# Autodesk Inventor assembly: MR126ZZ
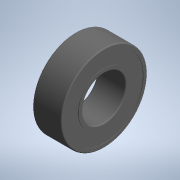
[picture p0: Inventor's stored thumbnail of the model, 180x180]
Saved by Autodesk Inventor 2022.3 (Build 263350000, 350)
## iProperties
Part Number: MR126ZZ
Catalog Web Link: www.cadenas.de
Description: Shielded Type ZZ-ZZS-
Vendor: NSK_RB
Document SubType Name: Assembly
Designer: partserver
Manufacturer: NSK_RB
Mass: 1.74 g
Surface Area: 9.09475 cm^2
Volume: 0.233443 cm^3
Density: 7.45365 g/cm^3
Category: PARTsolutions
Company: NSK_RB
PSOL_IDENT_0: {$CADENAS_DATA\23d-libs\nsk_rb\roller_bearings\deep_groove_bb\exstra_small_miniatur_bb\metric_design
PSOL_IDENT_1: \shielded_type_zz_zzs_asmtab.prj},174 {VTYP=3D},{STYP=ASSTAB},{NB=MR126ZZ},{LINA=MR126ZZ},{NN=Shield
PSOL_IDENT_2: ed Type ZZ-ZZS},{DATE=16.07.2021 00:25:30},{GEOMDATE=14.01.2008},{VERSION=},{LINEID=590},{WBVAR=},{W
PSOL_IDENT_3: BNUMERIC=}  {NB=MR126ZZ},{LINA=MR126ZZ},{KT=DUMMY},{IDNR=},{STAN=Standard},{ORDER=MR126ZZ},{SD=6.0},
PSOL_IDENT_4: {X=6.0},{DI1=7.73},{DI2=7.20},{SDE1=10.19},{SDE2=10.90},{D=12},{DD=12},{B=0.0},{B1=4.0},{R=0.00},{R1=
PSOL_IDENT_5: 0.15},{CR1=715},{COR1=292},{CR2=73},{COR2=30.0},{LG=43000},{LO=50000},{DA=0.0},{DB=7.2},{DA1=0.0},{D
PSOL_IDENT_6: B1=10.9},{RA=0.00},{RB=0.15},{MASS=1.74},{SC=1},{PPATH=shielded_type_zz_zzs_asmtpl.prj}
NB: MR126ZZ
NN: Shielded Type ZZ-ZZS
NBSYN: $ORDER.
LINA: MR126ZZ
CATALOG: NSK Rolling Bearing
STAN: Standard
ORDER: MR126ZZ
SD: 6
D: 12
B1: 4
R1: 0.15
CR1: 715
COR1: 292
CR2: 73
COR2: 30
LG: 43000
DB: 7.2
DB1: 10.9
RB: 0.15
MASS: 1.74
SUPPLIER: NSK_RB
ARTICLENO: MR126ZZ
BOMINFO: MR126ZZ
CREATOR: CADENAS GmbH
Title: MR126ZZ
Author: Cadenas PARTsolutions
## Documents named in this file (6)
- C:\Users\YusukeKunita\Documents\GrabCAD\Development\BasicParts\Bearing\NSK_RB_MR126ZZ\MR126ZZ.iam
- C:\Users\YusukeKunita\Documents\GrabCAD\Development\BasicParts\Bearing\NSK_RB_MR126ZZ\MR126ZZ Outer Ring.ipt
- C:\Users\YusukeKunita\Documents\GrabCAD\Development\BasicParts\Bearing\NSK_RB_MR126ZZ\MR126ZZ Inner Ring.ipt
- C:\Users\YusukeKunita\Documents\GrabCAD\Development\BasicParts\Bearing\NSK_RB_MR126ZZ\MR126ZZ Shield1.ipt
- C:\Users\YusukeKunita\Documents\GrabCAD\Development\BasicParts\Bearing\NSK_RB_MR126ZZ\MR126ZZ Ball.ipt
- C:\Users\YusukeKunita\Documents\GrabCAD\Development\BasicParts\Bearing\NSK_RB_MR126ZZ\MR126ZZ Shield2.ipt
## Components (16 placed, 5 different names)
1. MR126ZZ Outer Ring:1 — ip_st_or_1_XY@1 <-> ip_st_ir_1a_XY@2, ip_st_or_1_Z@1 <-> ip_st_ir_1a_Z@2, ip_st_or_1_YZ@1 <-> ip_st_ir_1a_YZ@2, ip_st_or_2_XY@1 <-> ip_st_s2_XY@16, ip_st_or_2_Z@1 <-> ip_st_s2_Z@16, ip_st_or_2_YZ@1 <-> ip_st_s2_YZ@16
2. MR126ZZ Inner Ring:1 — ip_st_or_1_XY@1 <-> ip_st_ir_1a_XY@2, ip_st_or_1_Z@1 <-> ip_st_ir_1a_Z@2, ip_st_or_1_YZ@1 <-> ip_st_ir_1a_YZ@2, ip_st_ir_2a_XY@2 <-> ip_st_s1_XY@3, ip_st_ir_2a_Z@2 <-> ip_st_s1_Z@3, ip_st_ir_2a_YZ@2 <-> ip_st_s1_YZ@3, ip_st_ir_1_1_XY@2 <-> ip_st_b_XY@4, ip_st_ir_1_1_Z@2 <-> ip_st_b_Z@4, ip_st_ir_1_1_YZ@2 <-> ip_st_b_YZ@4, ip_st_ir_1_2_XY@2 <-> ip_st_b_XY@5, ip_st_ir_1_2_Z@2 <-> ip_st_b_Z@5, ip_st_ir_1_2_YZ@2 <-> ip_st_b_YZ@5, ip_st_ir_1_3_XY@2 <-> ip_st_b_XY@6, ip_st_ir_1_3_Z@2 <-> ip_st_b_Z@6, ip_st_ir_1_3_YZ@2 <-> ip_st_b_YZ@6, ip_st_ir_1_4_XY@2 <-> ip_st_b_XY@7, ip_st_ir_1_4_Z@2 <-> ip_st_b_Z@7, ip_st_ir_1_4_YZ@2 <-> ip_st_b_YZ@7, ip_st_ir_1_5_XY@2 <-> ip_st_b_XY@8, ip_st_ir_1_5_Z@2 <-> ip_st_b_Z@8, ip_st_ir_1_5_YZ@2 <-> ip_st_b_YZ@8, ip_st_ir_1_6_XY@2 <-> ip_st_b_XY@9, ip_st_ir_1_6_Z@2 <-> ip_st_b_Z@9, ip_st_ir_1_6_YZ@2 <-> ip_st_b_YZ@9, ip_st_ir_1_7_XY@2 <-> ip_st_b_XY@10, ip_st_ir_1_7_Z@2 <-> ip_st_b_Z@10, ip_st_ir_1_7_YZ@2 <-> ip_st_b_YZ@10, ip_st_ir_1_8_XY@2 <-> ip_st_b_XY@11, ip_st_ir_1_8_Z@2 <-> ip_st_b_Z@11, ip_st_ir_1_8_YZ@2 <-> ip_st_b_YZ@11, ip_st_ir_1_9_XY@2 <-> ip_st_b_XY@12, ip_st_ir_1_9_Z@2 <-> ip_st_b_Z@12, ip_st_ir_1_9_YZ@2 <-> ip_st_b_YZ@12, ip_st_ir_1_10_XY@2 <-> ip_st_b_XY@13, ip_st_ir_1_10_Z@2 <-> ip_st_b_Z@13, ip_st_ir_1_10_YZ@2 <-> ip_st_b_YZ@13, ip_st_ir_1_11_XY@2 <-> ip_st_b_XY@14, ip_st_ir_1_11_Z@2 <-> ip_st_b_Z@14, ip_st_ir_1_11_YZ@2 <-> ip_st_b_YZ@14, ip_st_ir_1_12_XY@2 <-> ip_st_b_XY@15, ip_st_ir_1_12_Z@2 <-> ip_st_b_Z@15, ip_st_ir_1_12_YZ@2 <-> ip_st_b_YZ@15
3. MR126ZZ Shield1:1 — ip_st_ir_2a_XY@2 <-> ip_st_s1_XY@3, ip_st_ir_2a_Z@2 <-> ip_st_s1_Z@3, ip_st_ir_2a_YZ@2 <-> ip_st_s1_YZ@3
4. MR126ZZ Ball:1 — ip_st_ir_1_1_XY@2 <-> ip_st_b_XY@4, ip_st_ir_1_1_Z@2 <-> ip_st_b_Z@4, ip_st_ir_1_1_YZ@2 <-> ip_st_b_YZ@4
5. MR126ZZ Ball:2 — ip_st_ir_1_2_XY@2 <-> ip_st_b_XY@5, ip_st_ir_1_2_Z@2 <-> ip_st_b_Z@5, ip_st_ir_1_2_YZ@2 <-> ip_st_b_YZ@5
6. MR126ZZ Ball:3 — ip_st_ir_1_3_XY@2 <-> ip_st_b_XY@6, ip_st_ir_1_3_Z@2 <-> ip_st_b_Z@6, ip_st_ir_1_3_YZ@2 <-> ip_st_b_YZ@6
7. MR126ZZ Ball:4 — ip_st_ir_1_4_XY@2 <-> ip_st_b_XY@7, ip_st_ir_1_4_Z@2 <-> ip_st_b_Z@7, ip_st_ir_1_4_YZ@2 <-> ip_st_b_YZ@7
8. MR126ZZ Ball:5 — ip_st_ir_1_5_XY@2 <-> ip_st_b_XY@8, ip_st_ir_1_5_Z@2 <-> ip_st_b_Z@8, ip_st_ir_1_5_YZ@2 <-> ip_st_b_YZ@8
9. MR126ZZ Ball:6 — ip_st_ir_1_6_XY@2 <-> ip_st_b_XY@9, ip_st_ir_1_6_Z@2 <-> ip_st_b_Z@9, ip_st_ir_1_6_YZ@2 <-> ip_st_b_YZ@9
10. MR126ZZ Ball:7 — ip_st_ir_1_7_XY@2 <-> ip_st_b_XY@10, ip_st_ir_1_7_Z@2 <-> ip_st_b_Z@10, ip_st_ir_1_7_YZ@2 <-> ip_st_b_YZ@10
11. MR126ZZ Ball:8 — ip_st_ir_1_8_XY@2 <-> ip_st_b_XY@11, ip_st_ir_1_8_Z@2 <-> ip_st_b_Z@11, ip_st_ir_1_8_YZ@2 <-> ip_st_b_YZ@11
12. MR126ZZ Ball:9 — ip_st_ir_1_9_XY@2 <-> ip_st_b_XY@12, ip_st_ir_1_9_Z@2 <-> ip_st_b_Z@12, ip_st_ir_1_9_YZ@2 <-> ip_st_b_YZ@12
13. MR126ZZ Ball:10 — ip_st_ir_1_10_XY@2 <-> ip_st_b_XY@13, ip_st_ir_1_10_Z@2 <-> ip_st_b_Z@13, ip_st_ir_1_10_YZ@2 <-> ip_st_b_YZ@13
14. MR126ZZ Ball:11 — ip_st_ir_1_11_XY@2 <-> ip_st_b_XY@14, ip_st_ir_1_11_Z@2 <-> ip_st_b_Z@14, ip_st_ir_1_11_YZ@2 <-> ip_st_b_YZ@14
15. MR126ZZ Ball:12 — ip_st_ir_1_12_XY@2 <-> ip_st_b_XY@15, ip_st_ir_1_12_Z@2 <-> ip_st_b_Z@15, ip_st_ir_1_12_YZ@2 <-> ip_st_b_YZ@15
16. MR126ZZ Shield2:1 — ip_st_or_2_XY@1 <-> ip_st_s2_XY@16, ip_st_or_2_Z@1 <-> ip_st_s2_Z@16, ip_st_or_2_YZ@1 <-> ip_st_s2_YZ@16
## Relationships (45: Mate 29, Angle 15, Flush 1)
- ip_st_or_1_XY@1 <-> ip_st_ir_1a_XY@2 [Flush]: MR126ZZ Outer Ring:1 ↔ MR126ZZ Inner Ring:1
- ip_st_or_1_Z@1 <-> ip_st_ir_1a_Z@2 [Mate]: MR126ZZ Outer Ring:1 ↔ MR126ZZ Inner Ring:1
- ip_st_or_1_YZ@1 <-> ip_st_ir_1a_YZ@2 [Angle] (90 deg): MR126ZZ Outer Ring:1 ↔ MR126ZZ Inner Ring:1
- ip_st_ir_2a_XY@2 <-> ip_st_s1_XY@3 [Mate]: MR126ZZ Inner Ring:1 ↔ MR126ZZ Shield1:1
- ip_st_ir_2a_Z@2 <-> ip_st_s1_Z@3 [Mate]: MR126ZZ Inner Ring:1 ↔ MR126ZZ Shield1:1
- ip_st_ir_2a_YZ@2 <-> ip_st_s1_YZ@3 [Angle] (0 deg): MR126ZZ Inner Ring:1 ↔ MR126ZZ Shield1:1
- ip_st_ir_1_1_XY@2 <-> ip_st_b_XY@4 [Mate]: MR126ZZ Inner Ring:1 ↔ MR126ZZ Ball:1
- ip_st_ir_1_1_Z@2 <-> ip_st_b_Z@4 [Mate]: MR126ZZ Inner Ring:1 ↔ MR126ZZ Ball:1
- ip_st_ir_1_1_YZ@2 <-> ip_st_b_YZ@4 [Angle] (0 deg): MR126ZZ Inner Ring:1 ↔ MR126ZZ Ball:1
- ip_st_ir_1_2_XY@2 <-> ip_st_b_XY@5 [Mate]: MR126ZZ Inner Ring:1 ↔ MR126ZZ Ball:2
- ip_st_ir_1_2_Z@2 <-> ip_st_b_Z@5 [Mate]: MR126ZZ Inner Ring:1 ↔ MR126ZZ Ball:2
- ip_st_ir_1_2_YZ@2 <-> ip_st_b_YZ@5 [Angle] (0 deg): MR126ZZ Inner Ring:1 ↔ MR126ZZ Ball:2
- ip_st_ir_1_3_XY@2 <-> ip_st_b_XY@6 [Mate]: MR126ZZ Inner Ring:1 ↔ MR126ZZ Ball:3
- ip_st_ir_1_3_Z@2 <-> ip_st_b_Z@6 [Mate]: MR126ZZ Inner Ring:1 ↔ MR126ZZ Ball:3
- ip_st_ir_1_3_YZ@2 <-> ip_st_b_YZ@6 [Angle] (0 deg): MR126ZZ Inner Ring:1 ↔ MR126ZZ Ball:3
- ip_st_ir_1_4_XY@2 <-> ip_st_b_XY@7 [Mate]: MR126ZZ Inner Ring:1 ↔ MR126ZZ Ball:4
- ip_st_ir_1_4_Z@2 <-> ip_st_b_Z@7 [Mate]: MR126ZZ Inner Ring:1 ↔ MR126ZZ Ball:4
- ip_st_ir_1_4_YZ@2 <-> ip_st_b_YZ@7 [Angle] (0 deg): MR126ZZ Inner Ring:1 ↔ MR126ZZ Ball:4
- ip_st_ir_1_5_XY@2 <-> ip_st_b_XY@8 [Mate]: MR126ZZ Inner Ring:1 ↔ MR126ZZ Ball:5
- ip_st_ir_1_5_Z@2 <-> ip_st_b_Z@8 [Mate]: MR126ZZ Inner Ring:1 ↔ MR126ZZ Ball:5
- ip_st_ir_1_5_YZ@2 <-> ip_st_b_YZ@8 [Angle] (0 deg): MR126ZZ Inner Ring:1 ↔ MR126ZZ Ball:5
- ip_st_ir_1_6_XY@2 <-> ip_st_b_XY@9 [Mate]: MR126ZZ Inner Ring:1 ↔ MR126ZZ Ball:6
- ip_st_ir_1_6_Z@2 <-> ip_st_b_Z@9 [Mate]: MR126ZZ Inner Ring:1 ↔ MR126ZZ Ball:6
- ip_st_ir_1_6_YZ@2 <-> ip_st_b_YZ@9 [Angle] (0 deg): MR126ZZ Inner Ring:1 ↔ MR126ZZ Ball:6
- ip_st_ir_1_7_XY@2 <-> ip_st_b_XY@10 [Mate]: MR126ZZ Inner Ring:1 ↔ MR126ZZ Ball:7
- ip_st_ir_1_7_Z@2 <-> ip_st_b_Z@10 [Mate]: MR126ZZ Inner Ring:1 ↔ MR126ZZ Ball:7
- ip_st_ir_1_7_YZ@2 <-> ip_st_b_YZ@10 [Angle] (0 deg): MR126ZZ Inner Ring:1 ↔ MR126ZZ Ball:7
- ip_st_ir_1_8_XY@2 <-> ip_st_b_XY@11 [Mate]: MR126ZZ Inner Ring:1 ↔ MR126ZZ Ball:8
- ip_st_ir_1_8_Z@2 <-> ip_st_b_Z@11 [Mate]: MR126ZZ Inner Ring:1 ↔ MR126ZZ Ball:8
- ip_st_ir_1_8_YZ@2 <-> ip_st_b_YZ@11 [Angle] (0 deg): MR126ZZ Inner Ring:1 ↔ MR126ZZ Ball:8
- ip_st_ir_1_9_XY@2 <-> ip_st_b_XY@12 [Mate]: MR126ZZ Inner Ring:1 ↔ MR126ZZ Ball:9
- ip_st_ir_1_9_Z@2 <-> ip_st_b_Z@12 [Mate]: MR126ZZ Inner Ring:1 ↔ MR126ZZ Ball:9
- ip_st_ir_1_9_YZ@2 <-> ip_st_b_YZ@12 [Angle] (0 deg): MR126ZZ Inner Ring:1 ↔ MR126ZZ Ball:9
- ip_st_ir_1_10_XY@2 <-> ip_st_b_XY@13 [Mate]: MR126ZZ Inner Ring:1 ↔ MR126ZZ Ball:10
- ip_st_ir_1_10_Z@2 <-> ip_st_b_Z@13 [Mate]: MR126ZZ Inner Ring:1 ↔ MR126ZZ Ball:10
- ip_st_ir_1_10_YZ@2 <-> ip_st_b_YZ@13 [Angle] (0 deg): MR126ZZ Inner Ring:1 ↔ MR126ZZ Ball:10
- ip_st_ir_1_11_XY@2 <-> ip_st_b_XY@14 [Mate]: MR126ZZ Inner Ring:1 ↔ MR126ZZ Ball:11
- ip_st_ir_1_11_Z@2 <-> ip_st_b_Z@14 [Mate]: MR126ZZ Inner Ring:1 ↔ MR126ZZ Ball:11
- ip_st_ir_1_11_YZ@2 <-> ip_st_b_YZ@14 [Angle] (0 deg): MR126ZZ Inner Ring:1 ↔ MR126ZZ Ball:11
- ip_st_ir_1_12_XY@2 <-> ip_st_b_XY@15 [Mate]: MR126ZZ Inner Ring:1 ↔ MR126ZZ Ball:12
- ip_st_ir_1_12_Z@2 <-> ip_st_b_Z@15 [Mate]: MR126ZZ Inner Ring:1 ↔ MR126ZZ Ball:12
- ip_st_ir_1_12_YZ@2 <-> ip_st_b_YZ@15 [Angle] (0 deg): MR126ZZ Inner Ring:1 ↔ MR126ZZ Ball:12
- ip_st_or_2_XY@1 <-> ip_st_s2_XY@16 [Mate]: MR126ZZ Outer Ring:1 ↔ MR126ZZ Shield2:1
- ip_st_or_2_Z@1 <-> ip_st_s2_Z@16 [Mate]: MR126ZZ Outer Ring:1 ↔ MR126ZZ Shield2:1
- ip_st_or_2_YZ@1 <-> ip_st_s2_YZ@16 [Angle] (0 deg): MR126ZZ Outer Ring:1 ↔ MR126ZZ Shield2:1
